# Autodesk Inventor assembly: Wasp Wheel Assembly Left
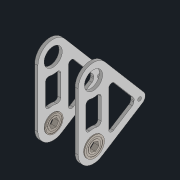
[picture p0: Inventor's stored thumbnail of the model, 180x180]
Saved by Autodesk Inventor 2022 (Build 260153000, 153)
## iProperties
Created: 2022-09-18
Part Number: Wasp Wheel Assembly Left
Document SubType Name: Assembly
Designer: robpl
Author: robpl
## Documents named in this file (3)
- C:\Users\robpl\Downloads\22-20220924T142245Z-001\WASP 23-9-22\Workspaces\Workspace\Wasp Wheel Assembly Left.iam
- C:\Users\robpl\Downloads\22-20220924T142245Z-001\WASP 23-9-22\Workspaces\Workspace\Wasp Wheel Plate.ipt
- C:\Users\robpl\Downloads\22-20220924T142245Z-001\WASP 23-9-22\Workspaces\Workspace\0.5 Flanged Hex Bearing (1.125 OD) (217-3875).ipt
## Components (4 placed, 2 different names)
1. Wasp Wheel Plate:1 — Mate:1, Mate:2, Mate:3, Mate:5, Mate:7
2. Wasp Wheel Plate:2 — Mate:1, Mate:2, Mate:3, Mate:4, Mate:6
3. 0.5 Flanged Hex Bearing (1.125 OD) (217-3875):1 — Mate:4, Mate:6
4. 0.5 Flanged Hex Bearing (1.125 OD) (217-3875):2 — Mate:5, Mate:7
## Relationships (7: Mate 7)
- Mate:1: Wasp Wheel Plate:1 ↔ Wasp Wheel Plate:2
- Mate:2: Wasp Wheel Plate:1 ↔ Wasp Wheel Plate:2
- Mate:3 (58.5 mm): Wasp Wheel Plate:1 ↔ Wasp Wheel Plate:2
- Mate:4: Wasp Wheel Plate:2 ↔ 0.5 Flanged Hex Bearing (1.125 OD) (217-3875):1
- Mate:5: Wasp Wheel Plate:1 ↔ 0.5 Flanged Hex Bearing (1.125 OD) (217-3875):2
- Mate:6: Wasp Wheel Plate:2 ↔ 0.5 Flanged Hex Bearing (1.125 OD) (217-3875):1
- Mate:7: Wasp Wheel Plate:1 ↔ 0.5 Flanged Hex Bearing (1.125 OD) (217-3875):2
